# Autodesk Inventor assembly: parts_assembled
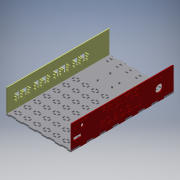
[picture p0: Inventor's stored thumbnail of the model, 180x180]
Saved by Autodesk Inventor 2016 (Build 200138000, 138)
## iProperties
Created: 2015-08-26
Part Number: parts_assembled
Document SubType Name: Assembly
Designer: gerthcm
Author: gerthcm
## Documents named in this file (4)
- C:\RobotCasserole\RoboSim\Enclosure_parts\parts_assembled.iam
- C:\RobotCasserole\RoboSim\Enclosure_parts\base.ipt
- C:\RobotCasserole\RoboSim\Enclosure_parts\front.ipt
- C:\RobotCasserole\RoboSim\Enclosure_parts\rear.ipt
## Components (3 placed, 3 different names)
1. base:1 — Mate:1, Mate:2, Mate:3, Mate:4, Mate:5, Mate:6
2. front:1 — Mate:1, Mate:2, Mate:3
3. rear:1 — Mate:4, Mate:5, Mate:6
## Relationships (6: Mate 6)
- Mate:1: base:1 ↔ front:1
- Mate:2: base:1 ↔ front:1
- Mate:3: base:1 ↔ front:1
- Mate:4: base:1 ↔ rear:1
- Mate:5: base:1 ↔ rear:1
- Mate:6: base:1 ↔ rear:1
